# Autodesk Inventor assembly: 316-03
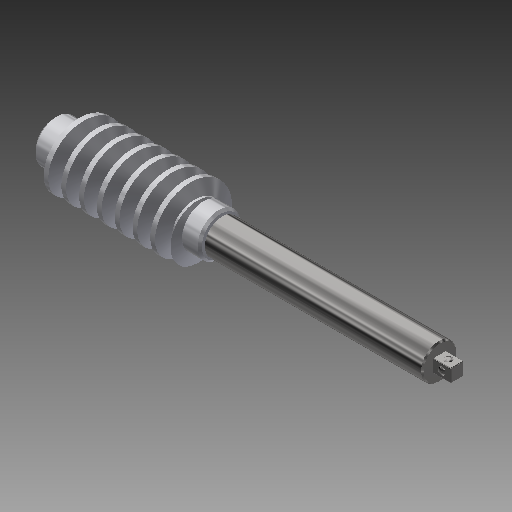
[picture p0: Inventor's stored thumbnail of the model, 512x512]
Saved by Autodesk Inventor 2019 (Build 230136000, 136)
## iProperties
Company: Autodesk Inc.
Created: 2008-01-21
Part Number: 316-03
Document SubType Name: Assembly
Designer: Autodesk Inc.
Mass: 26.1487 g
Surface Area: 46.9718 cm^2
Volume: 6.69385 cm^3
Density: 3.90639 g/cm^3
Author: Inventor
## Documents named in this file (3)
- C:\TEMP\Car Seat\Workspace\Worm Drive Shaft.iam
- C:\TEMP\Car Seat\Workspace\Worm Gear.ipt
- C:\TEMP\Car Seat\Workspace\Motor Connecting Rod.ipt
## Components (2 placed, 2 different names)
1. Motor Connecting Rod:1 — Insert:1
2. Worm:1 — Insert:1
## Relationships (1: Insert 1)
- Insert:1: Motor Connecting Rod:1 ↔ Worm:1
